# Autodesk Inventor assembly: BaseSuperior_final
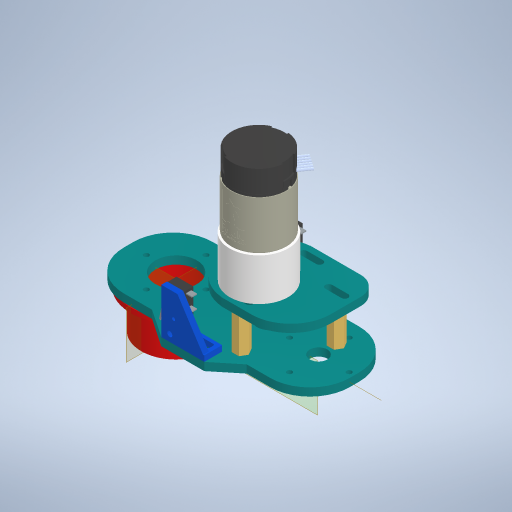
[picture p0: Inventor's stored thumbnail of the model, 512x512]
Saved by Autodesk Inventor 2024.3 (Build 283343000, 343)
## iProperties
Created: 2024-10-01
Part Number: BaseSuperior_final
Document SubType Name: Assembly
Designer: User
Author: User
## Documents named in this file (4)
- C:\Users\User\Documents\Universidad Octavo Semestre\Robotica Industrial\matlab\SCARA\mariana_scara_final\mariana_scara_final\BaseSuperior_final.iam
- C:\Users\User\Documents\Universidad Octavo Semestre\Robotica Industrial\matlab\SCARA\mariana_scara_final\mariana_scara_final\BaseSuperior.iam
- C:\Users\User\Documents\Universidad Octavo Semestre\Robotica Industrial\matlab\SCARA\mariana_scara_final\mariana_scara_final\soporterto_damiento.ipt
- C:\Users\User\Documents\Universidad Octavo Semestre\Robotica Industrial\matlab\SCARA\mariana_scara_final\mariana_scara_final\plea_peque.ipt
## Components (3 placed, 3 different names)
1. BaseSuperior:1 [sub-assembly] — Mate:1, Mate:2, Insert:1
2. soporterto_damiento:1 — Mate:1, Mate:2
3. plea_peque:1 — Insert:1
## Relationships (3: Mate 2, Insert 1)
- Mate:1: BaseSuperior:1 ↔ soporterto_damiento:1
- Mate:2: BaseSuperior:1 ↔ soporterto_damiento:1
- Insert:1: BaseSuperior:1 ↔ plea_peque:1
